# Autodesk Inventor assembly: 조립
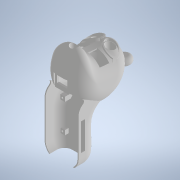
[picture p0: Inventor's stored thumbnail of the model, 180x180]
Saved by Autodesk Inventor 2022 (Build 260153000, 153)
## iProperties
Created: 2022-07-31
Part Number: 조립
Document SubType Name: Assembly
Designer: userpc
Author: userpc
## Documents named in this file (3)
- C:\Users\userpc\OneDrive\바탕 화면\다온\SSAFY\pjt\공통\조립.iam
- C:\Users\userpc\OneDrive\바탕 화면\다온\SSAFY\pjt\공통\0731_몸통.ipt
- C:\Users\userpc\OneDrive\바탕 화면\다온\SSAFY\pjt\공통\0730_얼굴.ipt
## Components (2 placed, 2 different names)
1. 0731_몸통:1 — 메이트:1
2. 0730_얼굴:1 — 플러쉬:2, 접선:1, 각도:1, 메이트:1
## Relationships (4: Flush 1, Tangent 1, Angle 1, Mate 1)
- 플러쉬:2 [Flush]: 0730_얼굴:1
- 접선:1 [Tangent] (-3 mm): 0730_얼굴:1
- 각도:1 [Angle] (90 deg): 0730_얼굴:1
- 메이트:1 [Mate]: 0731_몸통:1 ↔ 0730_얼굴:1
